# Autodesk Inventor assembly: LU15AL294K2720100W/O
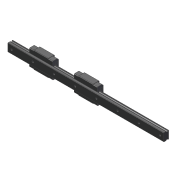
[picture p0: Inventor's stored thumbnail of the model, 180x180]
Saved by Autodesk Inventor 2015 (Build 190159000, 159)
## iProperties
Category: PARTsolutions
Company: NSK_RB
Created: 2015-07-20
Part Number: LU15AL294K2720100W/O
Catalog Web Link: www.cadenas.de
Description: LU15AL-
Vendor: NSK_RB
Document SubType Name: Assembly
Designer: PARTuser1
Manufacturer: NSK_RB
PSOL_IDENT_0: {$CADENAS_DATA\23d-libs\nsk_rb\nsk_linear_products\nsk_linear_guides\standard_series\lu_series\lu_al
PSOL_IDENT_1: _series\lu15al_asmtab.prj},209 {VTYP=3D},{STYP=ASSTAB},{NB=LU15AL294K2720100W/O},{LINA=LU15  294 AL
PSOL_IDENT_2: K 2},{NN=LU15AL},{DATE=18.06.2013 02:53:31},{GEOMDATE=27.05.2010},{VERSION=},{LINEID=740},{LINESUBID=
PSOL_IDENT_3: -1},{WBVAR=MAT,NOS,L0,G,POS1,POS2,SS}  {NB=LU15AL294K2720100W/O},{LINA=LU15  294 AL K 2},{KT=DUMMY},
PSOL_IDENT_4: {PN=LU15AL294K2720100W/O},{MN=LU15AL},{MNA=AL},{S=15},{MAT=K},{NOS=2},{L0=294},{G=7},{POS1=20},{POS2=
PSOL_IDENT_5: 100},{SS=W/O},{SSALG='W/O','Without Side seal'},{MAT1='C','Special High carbon steel', 'K','Stainles
PSOL_IDENT_6: s steel'},{H=16.0},{E=4.0},{W2=8.5},{W=32},{L=43.600},{B=25},{J=20},{M=3.0},{TL=4.0},{B1=3.5},{L1=27
PSOL_IDENT_7: .000},{J1=3.40},{K=12.0},{W1=15},{H1=9.5},{F=40},{D=3.500},{DD=6.000},{HH=4.500},{B3=7.5},{G1=15.0},
PSOL_IDENT_8: {GALGMIN=4},{GALGMAX=26.666667},{LMAX=1000},{LMIN=107.2},{NOMH=7},{POS1MIN=0},{POS1MAX=206.8},{POS2M
PSOL_IDENT_9: IN=63.6},{POS2MAX=250.4},{DT=3.5},{DDT=6},{HHT=4.5},{PPATH=parts/lu_asmtpl.prj}
SUPPLIER: NSK_RB
ARTICLENO: LU15AL294K2720100W/O
BOMINFO: LU15  294 AL K 2
CREATOR: CADENAS GmbH
Title: LU15  294 AL K 2
Author: Cadenas PARTsolutions
## Documents named in this file (4)
- C:\Dropbox\Inventor\Projects\Portalfraese_V2_Z-Axis\LU15AL294K2720100W_O.iam
- C:\Dropbox\Inventor\Projects\Portalfraese_V2_Z-Axis\LU15AL294K2720100_rail.ipt
- C:\Dropbox\Inventor\Projects\Portalfraese_V2_Z-Axis\LU15ALW_O_slider_1.ipt
- C:\Dropbox\Inventor\Projects\Portalfraese_V2_Z-Axis\LU15ALW_O_slider_2.ipt
## Components (3 placed, 3 different names)
1. LU15AL294K2720100_rail:1 — Mate:1, Mate:2, Mate:3, Mate:4
2. LU15ALW_O_slider_1:1 — Mate:3, Mate:4
3. LU15ALW_O_slider_2:1 — Mate:1, Mate:2
## Relationships (4: Mate 4)
- Mate:1: LU15AL294K2720100_rail:1 ↔ LU15ALW_O_slider_2:1
- Mate:2: LU15AL294K2720100_rail:1 ↔ LU15ALW_O_slider_2:1
- Mate:3: LU15AL294K2720100_rail:1 ↔ LU15ALW_O_slider_1:1
- Mate:4: LU15AL294K2720100_rail:1 ↔ LU15ALW_O_slider_1:1
